# Autodesk Inventor assembly: PCBBracket01
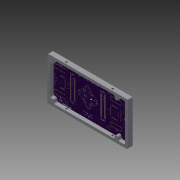
[picture p0: Inventor's stored thumbnail of the model, 180x180]
Saved by Autodesk Inventor 2015 (Build 190159000, 159)
## iProperties
Created: 2016-07-22
Part Number: PCBBracket01
Document SubType Name: Assembly
Designer: spichelh
Author: spichelh
## Documents named in this file (4)
- C:\Users\spichelh\Documents\GitHub\beta-hardware\Manufacturing Tools\PCB Reflow Bracket V01\PCBBracket01.iam
- C:\Users\spichelh\Documents\GitHub\beta-hardware\Manufacturing Tools\PCB Reflow Bracket V01\AXIOM Beta Mainboard.ipt
- C:\Users\spichelh\Documents\GitHub\beta-hardware\Manufacturing Tools\PCB Reflow Bracket V01\Bracket_TOP_V04.ipt
- C:\Users\spichelh\Documents\GitHub\beta-hardware\Manufacturing Tools\PCB Reflow Bracket V01\Bracket_BOT_V05.ipt
## Components (3 placed, 3 different names)
1. Bracket_BOT_V05:1 — Mate:2, Mate:3, Flush:1, Mate:12, Mate:13, Mate:14, Mate:16, Mate:17, Mate:18
2. AXIOM Beta Mainboard:1 — Mate:12, Mate:13, Mate:14
3. Bracket_TOP_V04:1 — Mate:16, Mate:17, Mate:18
## Relationships (9: Mate 8, Flush 1)
- Mate:2: Bracket_BOT_V05:1
- Mate:3: Bracket_BOT_V05:1
- Flush:1: Bracket_BOT_V05:1
- Mate:12: Bracket_BOT_V05:1 ↔ AXIOM Beta Mainboard:1
- Mate:13 (1 mm): Bracket_BOT_V05:1 ↔ AXIOM Beta Mainboard:1
- Mate:14 (1 mm): Bracket_BOT_V05:1 ↔ AXIOM Beta Mainboard:1
- Mate:16: Bracket_BOT_V05:1 ↔ Bracket_TOP_V04:1
- Mate:17: Bracket_BOT_V05:1 ↔ Bracket_TOP_V04:1
- Mate:18: Bracket_BOT_V05:1 ↔ Bracket_TOP_V04:1
